# Autodesk Inventor assembly: TURNBUCKLE,0.25IN_CLEVIS
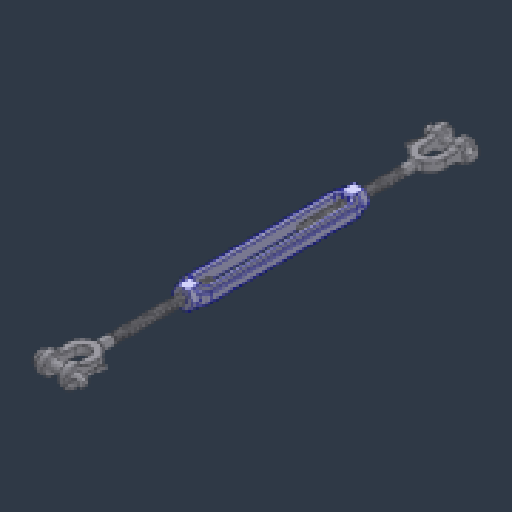
[picture p0: Inventor's stored thumbnail of the model, 512x512]
Saved by Autodesk Inventor 2024.3 (Build 283343000, 343)
## iProperties
Category: _
Manager: _
ILogicPurgeVersion: 0.0.0.0
OnSaveVersion: 3.4.3.0
OnSaveAssembly: COREAutomationManager
Created: 2025-01-30
Part Number: TURNBUCKLE,0.25IN_CLEVIS
Checked By: 00
Engr Approved By: _
User Status: Work In Process
Description: ASSY,STANDARD (mm)
Document SubType Name: Assembly
Mfg Approved By: John.Thibert
Designer: John.Thibert
Mass: 177.465 g
Surface Area: 175.676 cm^2
Volume: 22.3867 cm^3
CN_MASS: 0.18
CN_SERVICEABLE: _
FIRST_DESCRIPTION: _
SECOND_DESCRIPTION: _
THIRD_DESCRIPTION: _
CL_runCount: 0
ModelCat: Uncategorized
Subject: _
Author: John.Thibert
Keywords: -
Revision Number: A
## Documents named in this file (4)
- C:\Users\Johna\Documents\GitHub\2025-Poseidon-Mechanical\TURNBUCKLE,0.25IN_CLEVIS.iam
- C:\Users\Johna\Documents\GitHub\2025-Poseidon-Mechanical\3001T501.ipt
- C:\Users\Johna\Documents\GitHub\2025-Poseidon-Mechanical\3022T11_NO THREADS_316 Stainless Steel Turnbuckle-Not for Lift.ipt
- C:\Users\Johna\Documents\GitHub\2025-Poseidon-Mechanical\3001T701.ipt
## Components (3 placed, 3 different names)
1. 3022T11_NO THREADS_316 Stainless Steel Turnbuckle-Not for Lift.ipt:1 — Mate:1, Mate:2, Mate:4, Mate:7, Angle:1, Angle:3
2. 3001T501.ipt:1 — Mate:1, Mate:4, Mate:6, Angle:2
3. 3001T701.ipt:1 — Mate:2, Mate:3, Mate:6, Angle:2, Angle:3
## Relationships (9: Mate 6, Angle 3)
- Mate:1: 3022T11_NO THREADS_316 Stainless Steel Turnbuckle-Not for Lift.ipt:1 ↔ 3001T501.ipt:1
- Mate:2: 3022T11_NO THREADS_316 Stainless Steel Turnbuckle-Not for Lift.ipt:1 ↔ 3001T701.ipt:1
- Mate:3: 3001T701.ipt:1
- Mate:4 (9.525 mm): 3022T11_NO THREADS_316 Stainless Steel Turnbuckle-Not for Lift.ipt:1 ↔ 3001T501.ipt:1
- Mate:6: 3001T501.ipt:1 ↔ 3001T701.ipt:1
- Mate:7: 3022T11_NO THREADS_316 Stainless Steel Turnbuckle-Not for Lift.ipt:1
- Angle:1 (0 deg): 3022T11_NO THREADS_316 Stainless Steel Turnbuckle-Not for Lift.ipt:1
- Angle:2 (0 deg): 3001T501.ipt:1 ↔ 3001T701.ipt:1
- Angle:3 (0 deg): 3022T11_NO THREADS_316 Stainless Steel Turnbuckle-Not for Lift.ipt:1 ↔ 3001T701.ipt:1
